# Autodesk Inventor assembly: Передача с помощью зубчатых ремней
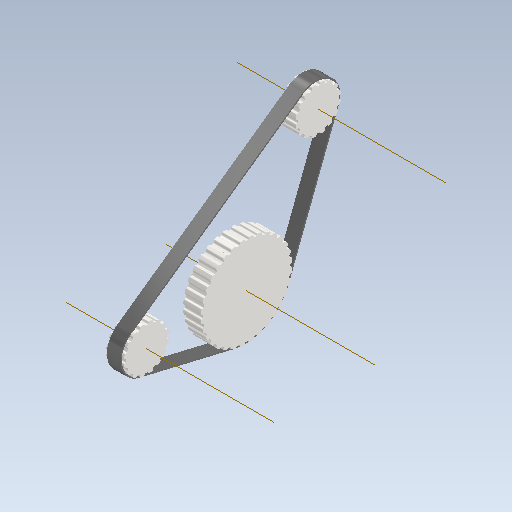
[picture p0: Inventor's stored thumbnail of the model, 512x512]
Saved by Autodesk Inventor 2021 (Build 250183000, 183)
## iProperties
ClientObjectVersion: 1
Created: 2021-06-16
Part Number: Передача с помощью зубчатых ремней
Document SubType Name: Assembly
Designer: panda
Author: panda
## Documents named in this file (5)
- C:\Users\panda\Desktop\vkrb\сборка\Сборка\Мастер проектирования\Передача с помощью зубчатых ремней6.iam
- C:\Users\panda\Desktop\vkrb\сборка\Сборка\Мастер проектирования\Зубчатый ремень6.ipt
- C:\Users\panda\Desktop\vkrb\сборка\Сборка\Мастер проектирования\Синхронный шкив15.ipt
- C:\Users\panda\Desktop\vkrb\сборка\Сборка\Мастер проектирования\Синхронный шкив26.ipt
- C:\Users\panda\Desktop\vkrb\сборка\Сборка\Мастер проектирования\Синхронный шкив34.ipt
## Components (4 placed, 4 different names)
1. Зубчатый ремень:1 — Заподлицо:1, Совмещение:1, Совмещение:2, Заподлицо:2, Совмещение:3, Совмещение:4, Заподлицо:3, Совмещение:5, Совмещение:6
2. Синхронный шкив1:1 — Заподлицо:1, Совмещение:1, Совмещение:2, ЗубчПер:1, ЗубчПер:2
3. Синхронный шкив2:1 — Заподлицо:2, Совмещение:3, ЗубчПер:1, Совмещение:4
4. Синхронный шкив3:1 — Заподлицо:3, Совмещение:5, ЗубчПер:2, Совмещение:6
## Relationships (11: Mate 6, Flush 3, RelateRotation 2)
- Заподлицо:1 [Flush]: Зубчатый ремень:1 ↔ Синхронный шкив1:1
- Совмещение:1 [Mate]: Зубчатый ремень:1 ↔ Синхронный шкив1:1
- Совмещение:2 [Mate]: Зубчатый ремень:1 ↔ Синхронный шкив1:1
- Заподлицо:2 [Flush]: Зубчатый ремень:1 ↔ Синхронный шкив2:1
- Совмещение:3 [Mate]: Зубчатый ремень:1 ↔ Синхронный шкив2:1
- ЗубчПер:1 [RelateRotation] (1 ul): Синхронный шкив1:1 ↔ Синхронный шкив2:1
- Совмещение:4 [Mate]: Зубчатый ремень:1 ↔ Синхронный шкив2:1
- Заподлицо:3 [Flush]: Зубчатый ремень:1 ↔ Синхронный шкив3:1
- Совмещение:5 [Mate]: Зубчатый ремень:1 ↔ Синхронный шкив3:1
- ЗубчПер:2 [RelateRotation] (2 ul): Синхронный шкив1:1 ↔ Синхронный шкив3:1
- Совмещение:6 [Mate]: Зубчатый ремень:1 ↔ Синхронный шкив3:1
